# Autodesk Inventor assembly: STL assembly
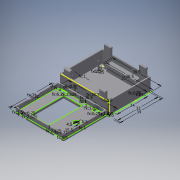
[picture p0: Inventor's stored thumbnail of the model, 180x180]
Saved by Autodesk Inventor 2019 (Build 230136000, 136)
## iProperties
Created: 2019-01-11
Part Number: STL assembly
Document SubType Name: Assembly
Designer: flato
Author: flato
## Documents named in this file (3)
- F:\Content creation\Projects\handheldWeatherStation\3D model\Inventor files\STL assembly.iam
- F:\Content creation\Projects\handheldWeatherStation\3D model\Inventor files\HandHeldWeatherStation housing.ipt
- F:\Content creation\Projects\handheldWeatherStation\3D model\Inventor files\Lid.ipt
## Components (2 placed, 2 different names)
1. Lid:1 — Mate:1, Flush:2
2. HandHeldWeatherStation housing:1 — Mate:2, Mate:3, Flush:3
## Relationships (5: Mate 3, Flush 2)
- Mate:1: Lid:1
- Mate:2: HandHeldWeatherStation housing:1
- Mate:3: HandHeldWeatherStation housing:1
- Flush:2: Lid:1
- Flush:3: HandHeldWeatherStation housing:1
